# Autodesk Inventor assembly: A_U_Boot
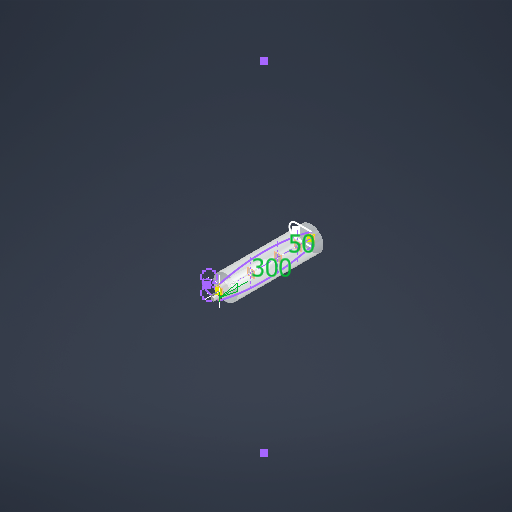
[picture p0: Inventor's stored thumbnail of the model, 512x512]
Saved by Autodesk Inventor 2026 (Build 300175000, 175)
## iProperties
Created: 2025-04-26
Part Number: A_U_Boot
Document SubType Name: Assembly
Designer: FAL
Author: FAL
## Documents named in this file (4)
- C:\Users\FAL\Desktop\git\U-BERT\CAD\A_U-Boot\A_U_Boot.iam
- C:\Users\FAL\Desktop\git\U-BERT\CAD\Trockenzelle\A_Trockenzelle.iam
- C:\Users\FAL\Desktop\git\U-BERT\CAD\Kolbentank\A_Kolbentank.iam
- C:\Users\FAL\Desktop\git\U-BERT\CAD\Rumpf\A_Rumpf.iam
## Components (3 placed, 3 different names)
1. A_Trockenzelle:1 [sub-assembly] — Fluchtend:1, Passend:1, Passend:2
2. A_Kolbentank:1 [sub-assembly] — Fluchtend:2, Passend:3
3. A_Rumpf:1 [sub-assembly] — Passend:4, Passend:5, Fluchtend:3
## Relationships (8: Mate 5, Flush 3)
- Fluchtend:1 [Flush]: A_Trockenzelle:1
- Passend:1 [Mate]: A_Trockenzelle:1
- Passend:2 [Mate]: A_Trockenzelle:1
- Fluchtend:2 [Flush]: A_Kolbentank:1
- Passend:3 [Mate]: A_Kolbentank:1
- Passend:4 [Mate]: A_Rumpf:1
- Passend:5 [Mate]: A_Rumpf:1
- Fluchtend:3 [Flush]: A_Rumpf:1
